# Autodesk Inventor assembly: ASY МОО 001 отстойник осветлитель
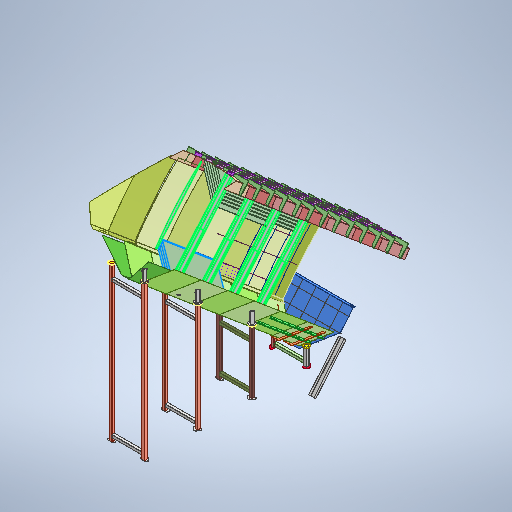
[picture p0: Inventor's stored thumbnail of the model, 512x512]
Saved by Autodesk Inventor 2025 (Build 290162010, 162A)
## iProperties
Created: 2024-04-28
Part Number: ASY МОО 001 отстойник осветлитель
Document SubType Name: Weldment
Designer: admin
Weld Material: Welded Aluminum-6061
Mass: 3.05393e+07 g
Surface Area: 3.06781e+06 cm^2
Volume: 2.84022e+07 cm^3
Density: 1.07525 g/cm^3
Author: admin
## Documents named in this file (68)
- C:\Users\user\YandexDisk\домашниий пк\Inventor\Manturovo\Manturovo_Se-clar\ASY MSC 001 отстойник осветлитель.iam
- C:\Users\user\YandexDisk\домашниий пк\Inventor\Manturovo\Manturovo_Se-clar\Рама основания\ASY MSC 090 base frame.iam
- C:\Users\user\YandexDisk\домашниий пк\Inventor\Manturovo\Manturovo_Se-clar\ASY MSC 080 roсket.iam
- C:\Users\user\YandexDisk\домашниий пк\Inventor\Manturovo\Manturovo_Se-clar\ASY MSC 010 cone.iam
- C:\Users\user\YandexDisk\домашниий пк\Inventor\Manturovo\Manturovo_Se-clar\MSC 000 DIM settler-clarifier.ipt
- C:\Users\user\YandexDisk\домашниий пк\Inventor\Manturovo\Manturovo_Se-clar\MSC 031 sheet lowerback.ipt
- C:\Users\user\YandexDisk\домашниий пк\Inventor\Manturovo\Manturovo_Se-clar\MSC 021 sheet left board hip.ipt
- C:\Users\user\YandexDisk\домашниий пк\Inventor\Manturovo\Manturovo_Se-clar\MSC 022 sheet right board hip.ipt
- C:\Users\user\YandexDisk\домашниий пк\Inventor\Manturovo\Manturovo_Se-clar\конус\MSC 071 ridge 1.ipt
- C:\Users\user\YandexDisk\домашниий пк\Inventor\Manturovo\Manturovo_Se-clar\конус\MSC 073 ridge 3.ipt
- C:\Users\user\YandexDisk\домашниий пк\Inventor\Manturovo\Manturovo_Se-clar\конус\MSC 074 face 1.ipt
- C:\Users\user\YandexDisk\домашниий пк\Inventor\Manturovo\Manturovo_Se-clar\Content Center Files\en-US\ISO 5251 B 3D\ISO 5251 Bends 3D without straight ends(90 deg) DN150 11 11.ipt
- C:\Users\user\YandexDisk\домашниий пк\Inventor\Manturovo\Manturovo_Se-clar\МОО 061 труба верх 1.ipt
- C:\Users\user\YandexDisk\домашниий пк\Inventor\Manturovo\Manturovo_Se-clar\МОО 062 труба верх 2.ipt
- C:\Users\user\YandexDisk\домашниий пк\Inventor\Manturovo\Manturovo_Se-clar\МОО 063 труба верх 3.ipt
- C:\Users\user\YandexDisk\домашниий пк\Inventor\Manturovo\Manturovo_Se-clar\Part1.ipt
- C:\Users\user\YandexDisk\домашниий пк\Inventor\Manturovo\Manturovo_Se-clar\MSC 0101 sheet gills.ipt
- C:\Users\user\YandexDisk\домашниий пк\Inventor\Manturovo\Manturovo_Se-clar\MSC 068 stringer lowerback.ipt
- C:\Users\user\YandexDisk\домашниий пк\Inventor\Manturovo\Manturovo_Se-clar\конус\MSC 072 ridge 2.ipt
- C:\Users\user\YandexDisk\домашниий пк\Inventor\Manturovo\Manturovo_Se-clar\MSC 075 face 2.ipt
- C:\Users\user\YandexDisk\домашниий пк\Inventor\Manturovo\Manturovo_Se-clar\MSC 076 face 3.ipt
- C:\Users\user\YandexDisk\домашниий пк\Inventor\Manturovo\Manturovo_Se-clar\MSC 077 face 4.ipt
- C:\Users\user\YandexDisk\домашниий пк\Inventor\Manturovo\Manturovo_Se-clar\MSC 035 ring.ipt
- C:\Users\user\YandexDisk\домашниий пк\Inventor\Manturovo\Manturovo_Se-clar\MSC 074 ridge 4.ipt
- C:\Users\user\YandexDisk\домашниий пк\Inventor\Manturovo\Manturovo_Se-clar\MSC 075 ridge 5.ipt
- C:\Users\user\YandexDisk\домашниий пк\Inventor\Manturovo\Manturovo_Se-clar\MSC 081 pillar 1.ipt
- C:\Users\user\YandexDisk\домашниий пк\Inventor\Manturovo\Manturovo_Se-clar\MSC 036 flange 500.ipt
- C:\Users\user\YandexDisk\домашниий пк\Inventor\Manturovo\Manturovo_Se-clar\MSC 037 flange cover 500.ipt
- C:\Users\user\YandexDisk\домашниий пк\Inventor\Manturovo\Manturovo_Se-clar\MSC 038 flange cover ring 500.ipt
- C:\Users\user\YandexDisk\домашниий пк\Inventor\Manturovo\Manturovo_Se-clar\MSC 039 flange cover plate 500.ipt
- C:\Users\user\YandexDisk\домашниий пк\Inventor\Manturovo\Manturovo_Se-clar\Рама основания\ASY MSC 120  base frame.iam
- C:\Users\user\YandexDisk\домашниий пк\Inventor\Manturovo\Manturovo_Se-clar\Рама основания\ASY MSC 121  base frame.iam
- C:\Users\user\YandexDisk\домашниий пк\Inventor\Manturovo\Manturovo_Se-clar\Чертеж для парам. рамы.ipt
- C:\Users\user\YandexDisk\домашниий пк\Inventor\Manturovo\Manturovo_Se-clar\ASY MSC 120.1  base frame.iam
- C:\Users\user\YandexDisk\домашниий пк\Inventor\Manturovo\Manturovo_Se-clar\ASY MSC 122  base frame.iam
- C:\Users\user\YandexDisk\домашниий пк\Inventor\Manturovo\Manturovo_Se-clar\ASY MSC 201 BACK.iam
- C:\Users\user\YandexDisk\домашниий пк\Inventor\Manturovo\Manturovo_Se-clar\ASY MSC 202 LEFT BOARD.iam
- C:\Users\user\YandexDisk\домашниий пк\Inventor\Manturovo\Manturovo_Se-clar\ASY MSC 203 RIGHT BOARD.iam
- C:\Users\user\YandexDisk\домашниий пк\Inventor\Manturovo\Manturovo_Se-clar\ASY MSC 204 BELLY.iam
- C:\Users\user\YandexDisk\домашниий пк\Inventor\Manturovo\Manturovo_Se-clar\MSC 063 stringer board #.ipt
- C:\Users\user\YandexDisk\домашниий пк\Inventor\Manturovo\Manturovo_Se-clar\MSC 064 stringer board ##.ipt
- C:\Users\user\YandexDisk\домашниий пк\Inventor\Manturovo\Manturovo_Se-clar\MSC 055 rib hip 2.ipt
- C:\Users\user\YandexDisk\домашниий пк\Inventor\Manturovo\Manturovo_Se-clar\MSC 054 rib hip 1.ipt
- C:\Users\user\YandexDisk\домашниий пк\Inventor\Manturovo\Manturovo_Se-clar\MSC 0102 sheet gills.ipt
- C:\Users\user\YandexDisk\домашниий пк\Inventor\Manturovo\Manturovo_Se-clar\MSC 078 creen pillar.iam
- C:\Users\user\YandexDisk\домашниий пк\Inventor\Manturovo\Manturovo_Se-clar\MSC 0202 sheet gills.ipt
- C:\Users\user\YandexDisk\домашниий пк\Inventor\Manturovo\Manturovo_Se-clar\MSC 0103 sheet gills.ipt
- C:\Users\user\YandexDisk\домашниий пк\Inventor\Manturovo\Manturovo_Se-clar\MSC 0203 sheet gills.ipt
- C:\Users\user\YandexDisk\домашниий пк\Inventor\Manturovo\Manturovo_Se-clar\MSC 0104 sheet gills.ipt
- C:\Users\user\YandexDisk\домашниий пк\Inventor\Manturovo\Manturovo_Se-clar\MSC 0204 sheet gills.ipt
- C:\Users\user\YandexDisk\домашниий пк\Inventor\Manturovo\Manturovo_Se-clar\MSC 0105 sheet gills.ipt
- C:\Users\user\YandexDisk\домашниий пк\Inventor\Manturovo\Manturovo_Se-clar\MSC 0205 sheet gills.ipt
- C:\Users\user\YandexDisk\домашниий пк\Inventor\Manturovo\Manturovo_Se-clar\MSC 0106 sheet gills.ipt
- C:\Users\user\YandexDisk\домашниий пк\Inventor\Manturovo\Manturovo_Se-clar\MSC 0206 sheet gills.ipt
- C:\Users\user\YandexDisk\домашниий пк\Inventor\Manturovo\Manturovo_Se-clar\MSC 0107 sheet gills.ipt
- C:\Users\user\YandexDisk\домашниий пк\Inventor\Manturovo\Manturovo_Se-clar\MSC 0207 sheet gills.ipt
- C:\Users\user\YandexDisk\домашниий пк\Inventor\Manturovo\Manturovo_Se-clar\MSC 079 creen pillar.ipt
- C:\Users\user\YandexDisk\домашниий пк\Inventor\Manturovo\Manturovo_Se-clar\ASY MSC 120 support.iam
- C:\Users\user\YandexDisk\домашниий пк\Inventor\Manturovo\Manturovo_Se-clar\ракета\МОО 065 ракета труба 5.ipt
- C:\Users\user\YandexDisk\домашниий пк\Inventor\Manturovo\Manturovo_Se-clar\ракета\МОО 066 ракета труба 6.ipt
- C:\Users\user\YandexDisk\домашниий пк\Inventor\Manturovo\Manturovo_Se-clar\ракета\МОО 067 ракета труба 7.ipt
- C:\Users\user\YandexDisk\домашниий пк\Inventor\Manturovo\Manturovo_Se-clar\ракета\МОО 068 ракета труба 8.ipt
- C:\Users\user\YandexDisk\домашниий пк\Inventor\Manturovo\Manturovo_Se-clar\MSC 0391 flange.ipt
- C:\Users\user\YandexDisk\домашниий пк\Inventor\Manturovo\Manturovo_Se-clar\ASY MSC 0130 cone exit back.iam
- C:\Users\user\YandexDisk\домашниий пк\Inventor\Manturovo\Manturovo_Se-clar\MSC DIM 085 tube belly.ipt
- C:\Users\user\YandexDisk\домашниий пк\Inventor\Manturovo\Manturovo_Se-clar\MSC 082 pillar 2.ipt
- C:\Users\user\YandexDisk\домашниий пк\Inventor\Manturovo\Manturovo_Se-clar\MSC 081 pillar 1_CPY.ipt
- C:\Users\user\YandexDisk\домашниий пк\Inventor\Manturovo\Manturovo_Se-clar\MSC 0211 string for sheets.ipt
## Components (111 placed, 69 different names)
1. MSC 000 DIM settler-clarifier.ipt:1
2. MSC 001 DIM frame.ipt:1 — Flush:94, Mate:95, Mate:97, Mate:99, Mate:100
3. ASY MSC 010 cone.iam:1 [sub-assembly] — Flush:22, Mate:16, Flush:28, Mate:65, Mate:78, Tangent:11, Flush:79, Mate:83, Flush:100, Cylindrical:11
4. ASY MSC 120 support:1 [sub-assembly] — Cylindrical:6
5. ASY MSC 120 support:2 [sub-assembly] — Cylindrical:7
6. ASY MSC 120 support:3 [sub-assembly] — Cylindrical:8
7. ASY MSC 120 support:4 [sub-assembly] — Cylindrical:9
8. MSC 078 creen pillar:1 [sub-assembly]
9. ASY MSC 204 BELLY:1 [sub-assembly] — Mate:141, Mate:143, Flush:101, Mate:146, Mate:147
10. ASY MSC 203 RIGHT BOARD:1 [sub-assembly] — Mate:140, Mate:141, Tangent:16, Flush:102
11. ASY MSC 202 LEFT BOARD:1 [sub-assembly] — Mate:142, Mate:143, Tangent:17, Flush:103
12. ASY MSC 201 BACK:1 [sub-assembly] — Mate:134, Tangent:16, Tangent:17
13. ASY MSC 122  base frame:2 [sub-assembly] — Flush:97, Mate:102, Cylindrical:9
14. ASY MSC 120.1  base frame:2 [sub-assembly] — Flush:96, Mate:100, Mate:101, Cylindrical:7
15. ASY MSC 121  base frame:1 [sub-assembly] — Mate:98, Flush:95, Mate:99, Cylindrical:8
16. ASY MSC 120  base frame:1 [sub-assembly] — Flush:93, Mate:97, Cylindrical:6, Cylindrical:10
17. ASY MSC 080 roсket.iam:1 [sub-assembly] — Flush:23
18. ASY MSC 090 base frame.iam:1 [sub-assembly] — Flush:19, Flush:21, Flush:100
19. MSC 031 sheet lowerback.ipt:1 — Mate:15, Mate:16, Tangent:10, Tangent:11, Tangent:12, Cylindrical:2, Rigid:185, Mate:134
20. MSC 021 sheet left board hip.ipt:1 — Flush:41, Mate:78
21. MSC 022 sheet right board hip.ipt:1 — Mate:30
22. MSC 071 ridge 1.ipt:1 — Mate:50, Rigid:211
23. MSC 073 ridge 3.ipt:1 — Rotational:6, Rigid:210, Rigid:211
24. MSC 072 ridge 2.ipt:1 — Rotational:6
25. MSC 077 face 4.ipt:1
26. MSC 074 ridge 4:1 — Rigid:210
27. MSC 075 ridge 5:1
28. MSC 074 face 1.ipt:1 — Rigid:156, Rigid:157, Flush:62, Rigid:159
29. МОО 061 труба верх 1.ipt:1 — Rigid:59, Rigid:159
30. ISO 5251 Bends 3D without straight ends(90 deg) DN150 11 11.ipt:1 — Rigid:59, Rotational:2
31. МОО 062 труба верх 2.ipt:1 — Rigid:156
32. МОО 063 труба верх 3.ipt:1 — Rigid:157
33. Part1.ipt:1
34. MSC 068 stringer lowerback.ipt:1 — Mate:65, Tangent:10
35. МОО 061 труба верх 1.ipt:2 — Rotational:2
36. MSC 075 face 2.ipt:1 — Flush:61
37. MSC 076 face 3.ipt:1 — Flush:76
38. MSC 068 stringer lowerback:2 — Mate:83, Tangent:12
39. MSC 035 ring:1 — Cylindrical:2, Rigid:185, Rigid:186
40. MSC 036 flange 500:1 — Rigid:175
41. MSC 036 flange 500:2 — Rigid:175, Rigid:176, Rigid:186
42. MSC 036 flange 500:3 — Rigid:176, Rigid:177, Mate:87
43. MSC 036 flange 500:4 — Rigid:177, Rotational:4
44. MSC 037 flange cover 500:1 — Rotational:4, Mate:87, Rigid:178, Mate:108
45. MSC 038 flange cover ring 500:1 — Rigid:178, Mate:109, Tangent:15
46. MSC 055 rib hip 2:2
47. MSC 063 stringer board #.ipt:2
48. MSC 064 stringer board ##.ipt:2
49. MSC 054 rib board hip 1:2
50. MSC 063 stringer board #.ipt:1
51. MSC 054 rib board hip 1:1
52. MSC 055 rib hip 2:1
53. MSC 064 stringer board ##.ipt:1
54. MSC 0102 sheet gills:1 — Rigid:197, Mate:124, Mate:144, Flush:104, Flush:110, Flush:111
55. MSC 0202 sheet gills:1 — Rigid:197
56. MSC 0103 sheet gills:1 — Rigid:199, Mate:123, Mate:124, Flush:104, Flush:105, Flush:110, Flush:112
57. MSC 0203 sheet gills:1 — Rigid:199
58. MSC 0104 sheet gills:1 — Rigid:201, Mate:122, Mate:123, Flush:105, Flush:107, Flush:112, Flush:113
59. MSC 0204 sheet gills:1 — Rigid:201
60. MSC 0105 sheet gills:1 — Rigid:203, Mate:121, Mate:122, Flush:107, Flush:108, Flush:113, Flush:114
61. MSC 0205 sheet gills:1 — Rigid:203
62. MSC 0106 sheet gills:1 — Rigid:205, Mate:120, Mate:121, Flush:108, Flush:109, Flush:114, Flush:115
63. MSC 0206 sheet gills:1 — Rigid:205
64. MSC 0107 sheet gills:1 — Rigid:206, Mate:120, Flush:109, Flush:115
65. MSC 0207 sheet gills:1 — Rigid:206
66. МОО 065 ракета труба 5:1 — Rigid:209, Rotational:8
67. МОО 066 ракета труба 6:1
68. МОО 067 ракета труба 7:1 — Rigid:209
69. МОО 068 ракета труба 8:1 — Cylindrical:11
70. ASY MSC 120 support:5 [sub-assembly] — Cylindrical:10
71. MSC 0391 flange:1 — Rotational:8
72. ASY MSC 0130 cone exit back:1 [sub-assembly] — Mate:140, Mate:142, Flush:101, Flush:102, Flush:103
73. MSC DIM 085 tube belly:1 — Mate:146, Mate:147, Mate:145
74. MSC 0101 sheet gills.ipt:1 — Mate:144, Flush:111
75. MSC 082 pillar 2:1
76. MSC 039 flange cover plate 500:1 — Mate:108, Mate:109, Tangent:15
77. MSC 039 flange cover plate 500:2
78. MSC 039 flange cover plate 500:3
79. MSC 039 flange cover plate 500:4
80. MSC 039 flange cover plate 500:5
81. MSC 039 flange cover plate 500:6
82. MSC 039 flange cover plate 500:7
83. MSC 039 flange cover plate 500:8
84. MSC 039 flange cover plate 500:9
85. MSC 039 flange cover plate 500:10
86. MSC 039 flange cover plate 500:11
87. MSC 039 flange cover plate 500:12
88. MSC 079 creen pillar:2 — Mate:148, Flush:117, Rotational:9
89. MSC 081 pillar 1:1 — Mate:145, Flush:116, Rigid:212, Mate:148, Rotational:10
90. MSC 081 pillar 1_CPY:1 — Rigid:212
91. MSC 079 creen pillar:3
92. MSC 081 pillar 1:2
93. MSC 081 pillar 1_CPY:2
94. MSC 079 creen pillar:4
95. MSC 081 pillar 1:3
96. MSC 081 pillar 1_CPY:3
97. MSC 079 creen pillar:5
98. MSC 081 pillar 1:4
99. MSC 081 pillar 1_CPY:4
100. MSC 0101 sheet gills:2 — Tangent:18, Tangent:19, Tangent:20
101. MSC 0211 string for sheets:2 — Rotational:9, Tangent:18, Tangent:19
102. MSC 0211 string for sheets:1 — Flush:117, Rotational:10, Tangent:20
103. MSC 0101 sheet gills:3
104. MSC 0211 string for sheets:3
105. MSC 0211 string for sheets:4
106. MSC 0101 sheet gills:4
107. MSC 0211 string for sheets:5
108. MSC 0211 string for sheets:6
109. MSC 0101 sheet gills:5
110. MSC 0211 string for sheets:7
111. MSC 0211 string for sheets:8
## Component patterns: (12 elements, first: MSC 039 flange cover plate 500:1), (4 elements, first: MSC 079 creen pillar:2 + MSC 081 pillar 1:1 + MSC 081 pillar 1_CPY:1), (4 elements, first: MSC 0101 sheet gills:2 + MSC 0211 string for sheets:2 + MSC 0211 string for sheets:1)
## Relationships (113: Mate 36, Flush 33, WeldJoint 22, Tangent 9, CylindricalJoint 7, RevoluteJoint 6)
- [Flush]: ASY MSC 201 BACK:1
- Flush:19: ASY MSC 090 base frame.iam:1
- Flush:21: ASY MSC 090 base frame.iam:1
- Flush:22: ASY MSC 010 cone.iam:1
- Flush:23: ASY MSC 080 roсket.iam:1
- Mate:15: MSC 031 sheet lowerback.ipt:1
- Mate:16: ASY MSC 010 cone.iam:1 ↔ MSC 031 sheet lowerback.ipt:1
- Flush:28: ASY MSC 010 cone.iam:1
- Flush:41: MSC 021 sheet left board hip.ipt:1
- Mate:30: MSC 022 sheet right board hip.ipt:1
- Mate:50 (200 mm): MSC 071 ridge 1.ipt:1
- Rigid:59 [WeldJoint]: МОО 061 труба верх 1.ipt:1 ↔ ISO 5251 Bends 3D without straight ends(90 deg) DN150 11 11.ipt:1
- Mate:65: ASY MSC 010 cone.iam:1 ↔ MSC 068 stringer lowerback.ipt:1
- [Mate]: ASY MSC 201 BACK:1 ↔ MSC 068 stringer lowerback.ipt:1
- Tangent:10: MSC 031 sheet lowerback.ipt:1 ↔ MSC 068 stringer lowerback.ipt:1
- Rotational:2 [RevoluteJoint]: ISO 5251 Bends 3D without straight ends(90 deg) DN150 11 11.ipt:1 ↔ МОО 061 труба верх 1.ipt:2
- Flush:61: MSC 075 face 2.ipt:1
- Rigid:156 [WeldJoint]: MSC 074 face 1.ipt:1 ↔ МОО 062 труба верх 2.ipt:1
- Rigid:157 [WeldJoint]: MSC 074 face 1.ipt:1 ↔ МОО 063 труба верх 3.ipt:1
- Flush:62: MSC 074 face 1.ipt:1
- Rigid:159 [WeldJoint] (-200 mm): MSC 074 face 1.ipt:1 ↔ МОО 061 труба верх 1.ipt:1
- Flush:76: MSC 076 face 3.ipt:1
- Mate:78: ASY MSC 010 cone.iam:1 ↔ MSC 021 sheet left board hip.ipt:1
- Tangent:11 (22 mm): ASY MSC 010 cone.iam:1 ↔ MSC 031 sheet lowerback.ipt:1
- Flush:79: ASY MSC 010 cone.iam:1
- Mate:83: ASY MSC 010 cone.iam:1 ↔ MSC 068 stringer lowerback:2
- [Mate]: ASY MSC 201 BACK:1 ↔ MSC 068 stringer lowerback:2
- Tangent:12: MSC 031 sheet lowerback.ipt:1 ↔ MSC 068 stringer lowerback:2
- Rigid:175 [WeldJoint]: MSC 036 flange 500:1 ↔ MSC 036 flange 500:2
- Rigid:176 [WeldJoint]: MSC 036 flange 500:2 ↔ MSC 036 flange 500:3
- Rigid:177 [WeldJoint]: MSC 036 flange 500:3 ↔ MSC 036 flange 500:4
- Cylindrical:2: MSC 031 sheet lowerback.ipt:1 ↔ MSC 035 ring:1
- Rotational:4 [RevoluteJoint]: MSC 036 flange 500:4 ↔ MSC 037 flange cover 500:1
- Mate:87: MSC 036 flange 500:3 ↔ MSC 037 flange cover 500:1
- Rigid:178 [WeldJoint]: MSC 037 flange cover 500:1 ↔ MSC 038 flange cover ring 500:1
- Flush:93 (-3 mm): ASY MSC 120  base frame:1
- [Mate]: ASY MSC 120  base frame:1
- Flush:94: MSC 001 DIM frame.ipt:1
- Mate:95: MSC 001 DIM frame.ipt:1
- Mate:97: MSC 001 DIM frame.ipt:1 ↔ ASY MSC 120  base frame:1
- Mate:98: ASY MSC 121  base frame:1
- Flush:95 (-3 mm): ASY MSC 121  base frame:1
- Mate:99: MSC 001 DIM frame.ipt:1 ↔ ASY MSC 121  base frame:1
- Flush:96 (-3 mm): ASY MSC 120.1  base frame:2
- Mate:100: MSC 001 DIM frame.ipt:1 ↔ ASY MSC 120.1  base frame:2
- Mate:101: ASY MSC 120.1  base frame:2
- Flush:97 (-3 mm): ASY MSC 122  base frame:2
- Mate:102: ASY MSC 122  base frame:2
- Rigid:185 [WeldJoint] (20 mm): MSC 031 sheet lowerback.ipt:1 ↔ MSC 035 ring:1
- Mate:108: MSC 037 flange cover 500:1 ↔ MSC 039 flange cover plate 500:1
- Mate:109: MSC 038 flange cover ring 500:1 ↔ MSC 039 flange cover plate 500:1
- Tangent:15: MSC 038 flange cover ring 500:1 ↔ MSC 039 flange cover plate 500:1
- Rigid:186 [WeldJoint]: MSC 035 ring:1 ↔ MSC 036 flange 500:2
- Rigid:197 [WeldJoint]: MSC 0102 sheet gills:1 ↔ MSC 0202 sheet gills:1
- Rigid:199 [WeldJoint]: MSC 0103 sheet gills:1 ↔ MSC 0203 sheet gills:1
- Rigid:201 [WeldJoint]: MSC 0104 sheet gills:1 ↔ MSC 0204 sheet gills:1
- Rigid:203 [WeldJoint]: MSC 0105 sheet gills:1 ↔ MSC 0205 sheet gills:1
- Rigid:205 [WeldJoint]: MSC 0106 sheet gills:1 ↔ MSC 0206 sheet gills:1
- Rigid:206 [WeldJoint]: MSC 0107 sheet gills:1 ↔ MSC 0207 sheet gills:1
- Mate:120 (50 mm): MSC 0106 sheet gills:1 ↔ MSC 0107 sheet gills:1
- Mate:121 (50 mm): MSC 0105 sheet gills:1 ↔ MSC 0106 sheet gills:1
- Mate:122 (50 mm): MSC 0104 sheet gills:1 ↔ MSC 0105 sheet gills:1
- Mate:123 (50 mm): MSC 0103 sheet gills:1 ↔ MSC 0104 sheet gills:1
- Mate:124 (50 mm): MSC 0102 sheet gills:1 ↔ MSC 0103 sheet gills:1
- [Mate]: ASY MSC 204 BELLY:1 ↔ ASY MSC 0130 cone exit back:1
- Flush:100: ASY MSC 010 cone.iam:1 ↔ ASY MSC 090 base frame.iam:1
- Cylindrical:6: ASY MSC 120 support:1 ↔ ASY MSC 120  base frame:1
- Cylindrical:7: ASY MSC 120 support:2 ↔ ASY MSC 120.1  base frame:2
- Cylindrical:8: ASY MSC 120 support:3 ↔ ASY MSC 121  base frame:1
- Cylindrical:9: ASY MSC 120 support:4 ↔ ASY MSC 122  base frame:2
- Mate:134: ASY MSC 201 BACK:1 ↔ MSC 031 sheet lowerback.ipt:1
- [WeldJoint]: ASY MSC 010 cone.iam:1 ↔ ASY MSC 0130 cone exit back:1
- [WeldJoint]: МОО 067 ракета труба 7:1 ↔ ASY MSC 0130 cone exit back:1
- Rigid:209 [WeldJoint]: МОО 065 ракета труба 5:1 ↔ МОО 067 ракета труба 7:1
- Cylindrical:10: ASY MSC 120  base frame:1 ↔ ASY MSC 120 support:5
- Rotational:6 [RevoluteJoint]: MSC 073 ridge 3.ipt:1 ↔ MSC 072 ridge 2.ipt:1
- Rigid:210 [WeldJoint]: MSC 073 ridge 3.ipt:1 ↔ MSC 074 ridge 4:1
- Rigid:211 [WeldJoint]: MSC 071 ridge 1.ipt:1 ↔ MSC 073 ridge 3.ipt:1
- Rotational:8 [RevoluteJoint]: МОО 065 ракета труба 5:1 ↔ MSC 0391 flange:1
- Cylindrical:11: ASY MSC 010 cone.iam:1 ↔ МОО 068 ракета труба 8:1
- Mate:140: ASY MSC 203 RIGHT BOARD:1 ↔ ASY MSC 0130 cone exit back:1
- Mate:141: ASY MSC 204 BELLY:1 ↔ ASY MSC 203 RIGHT BOARD:1
- Tangent:16: ASY MSC 203 RIGHT BOARD:1 ↔ ASY MSC 201 BACK:1
- Mate:142: ASY MSC 202 LEFT BOARD:1 ↔ ASY MSC 0130 cone exit back:1
- Mate:143: ASY MSC 204 BELLY:1 ↔ ASY MSC 202 LEFT BOARD:1
- Tangent:17: ASY MSC 202 LEFT BOARD:1 ↔ ASY MSC 201 BACK:1
- Flush:101: ASY MSC 204 BELLY:1 ↔ ASY MSC 0130 cone exit back:1
- Flush:102: ASY MSC 203 RIGHT BOARD:1 ↔ ASY MSC 0130 cone exit back:1
- Flush:103: ASY MSC 202 LEFT BOARD:1 ↔ ASY MSC 0130 cone exit back:1
- Mate:144 (50 mm): MSC 0102 sheet gills:1 ↔ MSC 0101 sheet gills.ipt:1
- Flush:104: MSC 0102 sheet gills:1 ↔ MSC 0103 sheet gills:1
- Flush:105: MSC 0103 sheet gills:1 ↔ MSC 0104 sheet gills:1
- Flush:107: MSC 0104 sheet gills:1 ↔ MSC 0105 sheet gills:1
- Flush:108: MSC 0105 sheet gills:1 ↔ MSC 0106 sheet gills:1
- Flush:109: MSC 0106 sheet gills:1 ↔ MSC 0107 sheet gills:1
- Flush:110: MSC 0102 sheet gills:1 ↔ MSC 0103 sheet gills:1
- Flush:111: MSC 0102 sheet gills:1 ↔ MSC 0101 sheet gills.ipt:1
- Flush:112: MSC 0103 sheet gills:1 ↔ MSC 0104 sheet gills:1
- Flush:113: MSC 0104 sheet gills:1 ↔ MSC 0105 sheet gills:1
- Flush:114: MSC 0105 sheet gills:1 ↔ MSC 0106 sheet gills:1
- Flush:115: MSC 0106 sheet gills:1 ↔ MSC 0107 sheet gills:1
- Mate:145: MSC DIM 085 tube belly:1 ↔ MSC 081 pillar 1:1
- Flush:116: MSC 081 pillar 1:1
- Mate:146 (3 mm): ASY MSC 204 BELLY:1 ↔ MSC DIM 085 tube belly:1
- Mate:147 (3 mm): ASY MSC 204 BELLY:1 ↔ MSC DIM 085 tube belly:1
- Rigid:212 [WeldJoint]: MSC 081 pillar 1:1 ↔ MSC 081 pillar 1_CPY:1
- Mate:148 (635 mm): MSC 079 creen pillar:2 ↔ MSC 081 pillar 1:1
- Flush:117: MSC 079 creen pillar:2 ↔ MSC 0211 string for sheets:1
- Rotational:9 [RevoluteJoint] (-5 mm): MSC 079 creen pillar:2 ↔ MSC 0211 string for sheets:2
- Rotational:10 [RevoluteJoint] (-5 mm): MSC 081 pillar 1:1 ↔ MSC 0211 string for sheets:1
- Tangent:18: MSC 0101 sheet gills:2 ↔ MSC 0211 string for sheets:2
- Tangent:19: MSC 0101 sheet gills:2 ↔ MSC 0211 string for sheets:2
- Tangent:20: MSC 0101 sheet gills:2 ↔ MSC 0211 string for sheets:1
## Named parameters: Бак_нахлест_фланца = 25 mm, Шаг_опор_по_баку = 2000 mm
